# Autodesk Inventor assembly: NOSS조립
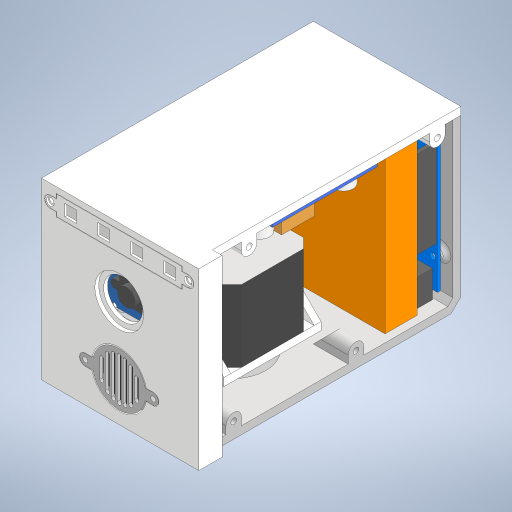
[picture p0: Inventor's stored thumbnail of the model, 512x512]
Saved by Autodesk Inventor 2023 (Build 270158000, 158)
## iProperties
Created: 2022-11-10
Part Number: NOSS조립
Document SubType Name: Assembly
Designer: user
Author: user
## Documents named in this file (13)
- C:\Users\user\Desktop\동국대 메이커톤\설계\NOSS조립.iam
- C:\Users\user\Desktop\동국대 메이커톤\설계\NOSS 하우징.ipt
- C:\Users\user\Desktop\동국대 메이커톤\설계\카메라 홀더.ipt
- C:\Users\user\Desktop\동국대 메이커톤\설계\제품 역설계\카메라.ipt
- C:\Users\user\Desktop\동국대 메이커톤\설계\제품 역설계\네오픽셀.ipt
- C:\Users\user\Desktop\동국대 메이커톤\설계\네오픽셀 홀더.ipt
- C:\Users\user\Desktop\동국대 메이커톤\설계\제품 역설계\스피커.ipt
- C:\Users\user\Desktop\동국대 메이커톤\설계\스피커 홀더.ipt
- C:\Users\user\Desktop\동국대 메이커톤\설계\제품 역설계\스텝모터 4401.ipt
- C:\Users\user\Desktop\동국대 메이커톤\설계\NOSS하단 커버.ipt
- C:\Users\user\Desktop\동국대 메이커톤\설계\제품 역설계\아두이노 우노.ipt
- C:\Users\user\Desktop\동국대 메이커톤\설계\제품 역설계\스텝다운 컨버터.ipt
- C:\Users\user\Desktop\동국대 메이커톤\설계\아크릴 커버.ipt
## Components (12 placed, 12 different names)
1. NOSS 하우징:1 — 삽입:5, 각도:1, 삽입:6, 삽입:7, 삽입:8, 삽입:11, 삽입:12, 삽입:13, 삽입:14, 메이트:4, 메이트:5, 삽입:18, 삽입:19, 삽입:20
2. 카메라 홀더:1 — 삽입:9, 삽입:10, 삽입:11, 삽입:12
3. 카메라:1 — 삽입:9, 삽입:10
4. 네오픽셀:1 — 메이트:1, 메이트:2, 메이트:3
5. 네오픽셀 홀더:1 — 메이트:1, 메이트:2, 메이트:3, 삽입:5, 각도:1
6. 스피커:1 — 삽입:6
7. 스피커 홀더:1 — 삽입:7, 삽입:8
8. 스텝모터 4401:1 — 삽입:13, 삽입:14
9. NOSS하단 커버:1 — 메이트:4, 메이트:5, 삽입:16, 삽입:17, 삽입:21
10. 아두이노 우노:1 — 삽입:16, 삽입:17
11. 스텝다운 컨버터:1 — 삽입:18, 삽입:19
12. 아크릴 커버:1 — 삽입:20, 삽입:21
## Relationships (22: Insert 16, Mate 5, Angle 1)
- 메이트:1 [Mate] (0.5 mm): 네오픽셀:1 ↔ 네오픽셀 홀더:1
- 메이트:2 [Mate] (0.5 mm): 네오픽셀:1 ↔ 네오픽셀 홀더:1
- 메이트:3 [Mate]: 네오픽셀:1 ↔ 네오픽셀 홀더:1
- 삽입:5 [Insert] (0.5 mm): NOSS 하우징:1 ↔ 네오픽셀 홀더:1
- 각도:1 [Angle] (180 deg): NOSS 하우징:1 ↔ 네오픽셀 홀더:1
- 삽입:6 [Insert]: NOSS 하우징:1 ↔ 스피커:1
- 삽입:7 [Insert]: NOSS 하우징:1 ↔ 스피커 홀더:1
- 삽입:8 [Insert]: NOSS 하우징:1 ↔ 스피커 홀더:1
- 삽입:9 [Insert]: 카메라 홀더:1 ↔ 카메라:1
- 삽입:10 [Insert]: 카메라 홀더:1 ↔ 카메라:1
- 삽입:11 [Insert]: NOSS 하우징:1 ↔ 카메라 홀더:1
- 삽입:12 [Insert]: NOSS 하우징:1 ↔ 카메라 홀더:1
- 삽입:13 [Insert]: NOSS 하우징:1 ↔ 스텝모터 4401:1
- 삽입:14 [Insert]: NOSS 하우징:1 ↔ 스텝모터 4401:1
- 메이트:4 [Mate]: NOSS 하우징:1 ↔ NOSS하단 커버:1
- 메이트:5 [Mate]: NOSS 하우징:1 ↔ NOSS하단 커버:1
- 삽입:16 [Insert]: NOSS하단 커버:1 ↔ 아두이노 우노:1
- 삽입:17 [Insert]: NOSS하단 커버:1 ↔ 아두이노 우노:1
- 삽입:18 [Insert]: NOSS 하우징:1 ↔ 스텝다운 컨버터:1
- 삽입:19 [Insert]: NOSS 하우징:1 ↔ 스텝다운 컨버터:1
- 삽입:20 [Insert]: NOSS 하우징:1 ↔ 아크릴 커버:1
- 삽입:21 [Insert]: NOSS하단 커버:1 ↔ 아크릴 커버:1
